# Autodesk Inventor assembly: 본체 조립
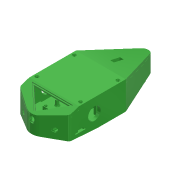
[picture p0: Inventor's stored thumbnail of the model, 180x180]
Saved by Autodesk Inventor 2020 (Build 240168000, 168)
## iProperties
Created: 2020-06-01
Part Number: 본체 조립
Document SubType Name: Assembly
Designer: Miji
Author: Miji
## Documents named in this file (8)
- C:\Users\82102\OneDrive\바탕 화면\개인자료\졸업과제\설계\로봇\모델링 1.2\본체 조립.iam
- C:\Users\82102\OneDrive\바탕 화면\개인자료\졸업과제\설계\로봇\모델링 1.2\본체 하단.ipt
- C:\Users\82102\OneDrive\바탕 화면\개인자료\졸업과제\설계\로봇\모델링 1.2\본체 커버.ipt
- C:\Users\82102\OneDrive\바탕 화면\개인자료\졸업과제\설계\로봇\모델링 1.2\볼캐스터.ipt
- C:\Users\82102\OneDrive\바탕 화면\개인자료\졸업과제\설계\로봇\모델링 1.2\모터 커버.ipt
- C:\Users\82102\OneDrive\바탕 화면\개인자료\졸업과제\설계\로봇\모델링 1.2\건전지 커버.ipt
- C:\Users\82102\OneDrive\바탕 화면\개인자료\졸업과제\설계\로봇\모델링 1.2\지름 모터 커버.ipt
- C:\Users\82102\OneDrive\바탕 화면\개인자료\졸업과제\설계\로봇\모델링 1.2\규격품\볼트 3M 6L.ipt
## Components (19 placed, 7 different names)
1. 본체 하단:1 — 메이트:1, 메이트:2, 메이트:6, 메이트:7, 메이트:8, 메이트:9, 메이트:10, 메이트:11, 메이트:12, 메이트:13, 메이트:14, 메이트:15, 메이트:16
2. 본체 커버:1 — 메이트:1, 메이트:2, 메이트:17, 메이트:18, 메이트:19, 메이트:20, 메이트:21, 각도:1
3. 볼캐스터:1 — 메이트:3, 메이트:4, 메이트:5, 메이트:7
4. 볼캐스터:2 — 메이트:3, 메이트:4, 메이트:5, 메이트:6
5. 모터 커버:1 — 메이트:8, 메이트:9, 메이트:10, 메이트:24, 메이트:26, 메이트:27, 메이트:28, 메이트:31
6. 건전지 커버:1 — 메이트:11, 메이트:12, 메이트:13
7. 지름 모터 커버:1 — 메이트:14, 메이트:15, 메이트:16, 메이트:22, 메이트:23, 메이트:25, 메이트:29, 메이트:30
8. 볼트 3M 6L:1 — 메이트:17, 메이트:18, 플러쉬:1, 플러쉬:2, 플러쉬:3, 각도:1, 각도:2
9. 볼트 3M 6L:2 — 메이트:19, 플러쉬:1, 각도:2, 각도:3
10. 볼트 3M 6L:3 — 메이트:20, 플러쉬:3, 각도:3, 각도:4
11. 볼트 3M 6L:4 — 메이트:21, 플러쉬:2, 각도:4, 각도:12
12. 볼트 3M 6L:5 — 메이트:22, 각도:10, 각도:11, 플러쉬:4, 플러쉬:5
13. 볼트 3M 6L:6 — 메이트:23, 각도:9, 각도:10, 플러쉬:5, 플러쉬:6, 메이트:30
14. 볼트 3M 6L:7 — 메이트:25, 각도:11, 플러쉬:4
15. 볼트 3M 6L:8 — 메이트:24, 각도:6, 각도:7, 각도:8, 플러쉬:8, 플러쉬:9, 각도:12
16. 볼트 3M 6L:9 — 메이트:26, 각도:5, 각도:6, 플러쉬:7, 플러쉬:9, 메이트:31
17. 볼트 3M 6L:10 — 메이트:27, 각도:5, 플러쉬:7
18. 볼트 3M 6L:11 — 메이트:28, 각도:7, 플러쉬:8
19. 볼트 3M 6L:12 — 메이트:29, 각도:8, 각도:9, 플러쉬:6
## Relationships (52: Mate 31, Angle 12, Flush 9)
- 메이트:1 [Mate]: 본체 하단:1 ↔ 본체 커버:1
- 메이트:2 [Mate]: 본체 하단:1 ↔ 본체 커버:1
- 메이트:3 [Mate]: 볼캐스터:1 ↔ 볼캐스터:2
- 메이트:4 [Mate]: 볼캐스터:1 ↔ 볼캐스터:2
- 메이트:5 [Mate]: 볼캐스터:1 ↔ 볼캐스터:2
- 메이트:6 [Mate]: 본체 하단:1 ↔ 볼캐스터:2
- 메이트:7 [Mate]: 본체 하단:1 ↔ 볼캐스터:1
- 메이트:8 [Mate]: 본체 하단:1 ↔ 모터 커버:1
- 메이트:9 [Mate]: 본체 하단:1 ↔ 모터 커버:1
- 메이트:10 [Mate]: 본체 하단:1 ↔ 모터 커버:1
- 메이트:11 [Mate]: 본체 하단:1 ↔ 건전지 커버:1
- 메이트:12 [Mate]: 본체 하단:1 ↔ 건전지 커버:1
- 메이트:13 [Mate]: 본체 하단:1 ↔ 건전지 커버:1
- 메이트:14 [Mate]: 본체 하단:1 ↔ 지름 모터 커버:1
- 메이트:15 [Mate]: 본체 하단:1 ↔ 지름 모터 커버:1
- 메이트:16 [Mate]: 본체 하단:1 ↔ 지름 모터 커버:1
- 메이트:17 [Mate]: 본체 커버:1 ↔ 볼트 3M 6L:1
- 메이트:18 [Mate]: 본체 커버:1 ↔ 볼트 3M 6L:1
- 메이트:19 [Mate]: 본체 커버:1 ↔ 볼트 3M 6L:2
- 플러쉬:1 [Flush]: 볼트 3M 6L:1 ↔ 볼트 3M 6L:2
- 메이트:20 [Mate]: 본체 커버:1 ↔ 볼트 3M 6L:3
- 메이트:21 [Mate]: 본체 커버:1 ↔ 볼트 3M 6L:4
- 플러쉬:2 [Flush]: 볼트 3M 6L:1 ↔ 볼트 3M 6L:4
- 플러쉬:3 [Flush]: 볼트 3M 6L:1 ↔ 볼트 3M 6L:3
- 각도:1 [Angle] (0 deg): 본체 커버:1 ↔ 볼트 3M 6L:1
- 각도:2 [Angle] (0 deg): 볼트 3M 6L:1 ↔ 볼트 3M 6L:2
- 각도:3 [Angle] (0 deg): 볼트 3M 6L:2 ↔ 볼트 3M 6L:3
- 각도:4 [Angle] (0 deg): 볼트 3M 6L:3 ↔ 볼트 3M 6L:4
- 메이트:22 [Mate]: 지름 모터 커버:1 ↔ 볼트 3M 6L:5
- 메이트:23 [Mate]: 지름 모터 커버:1 ↔ 볼트 3M 6L:6
- 메이트:24 [Mate]: 모터 커버:1 ↔ 볼트 3M 6L:8
- 메이트:25 [Mate]: 지름 모터 커버:1 ↔ 볼트 3M 6L:7
- 메이트:26 [Mate]: 모터 커버:1 ↔ 볼트 3M 6L:9
- 메이트:27 [Mate]: 모터 커버:1 ↔ 볼트 3M 6L:10
- 메이트:28 [Mate]: 모터 커버:1 ↔ 볼트 3M 6L:11
- 메이트:29 [Mate]: 지름 모터 커버:1 ↔ 볼트 3M 6L:12
- 각도:5 [Angle] (0 deg): 볼트 3M 6L:9 ↔ 볼트 3M 6L:10
- 각도:6 [Angle] (0 deg): 볼트 3M 6L:8 ↔ 볼트 3M 6L:9
- 각도:7 [Angle] (0 deg): 볼트 3M 6L:8 ↔ 볼트 3M 6L:11
- 각도:8 [Angle] (0 deg): 볼트 3M 6L:8 ↔ 볼트 3M 6L:12
- 각도:9 [Angle] (0 deg): 볼트 3M 6L:6 ↔ 볼트 3M 6L:12
- 각도:10 [Angle] (0 deg): 볼트 3M 6L:5 ↔ 볼트 3M 6L:6
- 각도:11 [Angle] (0 deg): 볼트 3M 6L:5 ↔ 볼트 3M 6L:7
- 플러쉬:4 [Flush]: 볼트 3M 6L:5 ↔ 볼트 3M 6L:7
- 플러쉬:5 [Flush]: 볼트 3M 6L:5 ↔ 볼트 3M 6L:6
- 플러쉬:6 [Flush]: 볼트 3M 6L:6 ↔ 볼트 3M 6L:12
- 메이트:30 [Mate] (0.7 mm): 지름 모터 커버:1 ↔ 볼트 3M 6L:6
- 플러쉬:7 [Flush]: 볼트 3M 6L:9 ↔ 볼트 3M 6L:10
- 플러쉬:8 [Flush]: 볼트 3M 6L:8 ↔ 볼트 3M 6L:11
- 플러쉬:9 [Flush]: 볼트 3M 6L:8 ↔ 볼트 3M 6L:9
- 메이트:31 [Mate] (-0.7 mm): 모터 커버:1 ↔ 볼트 3M 6L:9
- 각도:12 [Angle] (0 deg): 볼트 3M 6L:4 ↔ 볼트 3M 6L:8
